# Autodesk Inventor assembly: Cadena
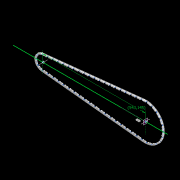
[picture p0: Inventor's stored thumbnail of the model, 180x180]
Saved by Autodesk Inventor 2021 (Build 250183000, 183)
## iProperties
Created: 2021-04-23
Part Number: Cadena
Document SubType Name: Assembly
Designer: maaro
Author: maaro
## Documents named in this file (4)
- C:\Users\maaro\Documents\UNAL\Automatización de Procesos de Manufactura\Github\Proyecto_APM\02 Inventor\Transmision\Cadena.iam
- C:\Users\maaro\Documents\UNAL\Automatización de Procesos de Manufactura\Github\Proyecto_APM\02 Inventor\Transmision\Design Accelerator\Roller Chain1.ipt
- C:\Users\maaro\Documents\UNAL\Automatización de Procesos de Manufactura\Github\Proyecto_APM\02 Inventor\Transmision\Eslabón 1.ipt
- C:\Users\maaro\Documents\UNAL\Automatización de Procesos de Manufactura\Github\Proyecto_APM\02 Inventor\Transmision\Eslabón 2.ipt
## Components (56 placed, 3 different names)
1. Roller Chain:1 — Flush:1, Flush:2, Flush:3, Mate:1, Mate:2, Angle:1
2. Eslabón 2:1
3. Eslabón 1:1 — Mate:1, Mate:2, Angle:1
4. Eslabón 1:2
5. Eslabón 1:3
6. Eslabón 1:4
7. Eslabón 1:5
8. Eslabón 1:6
9. Eslabón 1:7
10. Eslabón 1:8
11. Eslabón 1:9
12. Eslabón 1:10
13. Eslabón 1:11
14. Eslabón 1:12
15. Eslabón 1:13
16. Eslabón 1:14
17. Eslabón 1:15
18. Eslabón 1:16
19. Eslabón 1:17
20. Eslabón 1:18
21. Eslabón 1:19
22. Eslabón 1:20
23. Eslabón 1:21
24. Eslabón 1:22
25. Eslabón 1:23
26. Eslabón 1:24
27. Eslabón 1:25
28. Eslabón 1:26
29. Eslabón 1:27
30. Eslabón 1:28
31. Eslabón 1:29
32. Eslabón 1:30
33. Eslabón 1:31
34. Eslabón 1:32
35. Eslabón 1:33
36. Eslabón 1:34
37. Eslabón 1:35
38. Eslabón 1:36
39. Eslabón 1:37
40. Eslabón 1:38
41. Eslabón 1:39
42. Eslabón 1:40
43. Eslabón 1:41
44. Eslabón 1:42
45. Eslabón 1:43
46. Eslabón 1:44
47. Eslabón 1:45
48. Eslabón 1:46
49. Eslabón 1:47
50. Eslabón 1:48
51. Eslabón 1:49
52. Eslabón 1:50
53. Eslabón 1:51
54. Eslabón 1:52
55. Eslabón 1:53
56. Eslabón 1:54
## Component patterns: (54 elements, first: Eslabón 1:1)
## Relationships (6: Flush 3, Mate 2, Angle 1)
- Flush:1: Roller Chain:1
- Flush:2: Roller Chain:1
- Flush:3: Roller Chain:1
- Mate:1: Roller Chain:1 ↔ Eslabón 1:1
- Mate:2: Roller Chain:1 ↔ Eslabón 1:1
- Angle:1 (0 deg): Roller Chain:1 ↔ Eslabón 1:1
## Named parameters: start = 543.1451 mm
